# Autodesk Inventor assembly: ServoAssembly
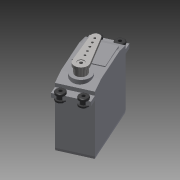
[picture p0: Inventor's stored thumbnail of the model, 180x180]
Saved by Autodesk Inventor 2015 (Build 190159000, 159)
## iProperties
Created: 2014-02-25
Part Number: ServoAssembly
Document SubType Name: Assembly
Designer: Jonathan
Author: Jonathan
## Documents named in this file (4)
- D:\Documents\GitHub\SolidModels\stag_v2_01_pre_alpha\ServoAssembly.iam
- D:\Documents\GitHub\SolidModels\stag_v2_01_pre_alpha\ServoModel.ipt
- D:\Documents\GitHub\SolidModels\stag_v2_01_pre_alpha\ServoHorn.ipt
- D:\Documents\GitHub\SolidModels\stag_v2_01_pre_alpha\Grommet.ipt
## Components (6 placed, 3 different names)
1. ServoModel:1 — Mate:1, Mate:2, Mate:3, Mate:4, Mate:5, Mate:6, Mate:7, Mate:8, Mate:9, Mate:10
2. ServoHorn:1 — Mate:1, Mate:2
3. Grommet:1 — Mate:3, Mate:4
4. Grommet:2 — Mate:5, Mate:6
5. Grommet:3 — Mate:7, Mate:8
6. Grommet:4 — Mate:9, Mate:10
## Relationships (10: Mate 10)
- Mate:1: ServoModel:1 ↔ ServoHorn:1
- Mate:2: ServoModel:1 ↔ ServoHorn:1
- Mate:3: ServoModel:1 ↔ Grommet:1
- Mate:4: ServoModel:1 ↔ Grommet:1
- Mate:5: ServoModel:1 ↔ Grommet:2
- Mate:6: ServoModel:1 ↔ Grommet:2
- Mate:7: ServoModel:1 ↔ Grommet:3
- Mate:8: ServoModel:1 ↔ Grommet:3
- Mate:9: ServoModel:1 ↔ Grommet:4
- Mate:10: ServoModel:1 ↔ Grommet:4
